# Autodesk Inventor assembly: M178-0001
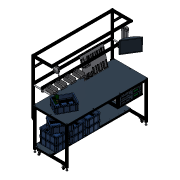
[picture p0: Inventor's stored thumbnail of the model, 180x180]
Saved by Autodesk Inventor 2018.3 (Build 223284000, 284)
## iProperties
Created: 2004-11-17
Part Number: M178-0001
Document SubType Name: Assembly
Designer: Autodesk, Inc.
Manufacturer: Standard
Standards Organization: Custom
Description: TEST STATION, STANDARD
Mass: 86518 g
Surface Area: 222281 cm^2
Volume: 49426.1 cm^3
Density: 1.75045 g/cm^3
Company: Autodesk, Inc.
Author: Autodesk, Inc.
CAGE: 1LJX3
Dept. ID: Product Design
Description #2: ---
Finish #1: ---
Finish #2: ---
Material ID: ---
Project Number: ---
## iProperties of the stored document _VirtualPart2
Created: 2006-02-28
Designer: Autodesk, Inc
Part Number: M178-S002
Description: TEST STATION SERVER SOFTWARE
Engineer: N. GINEER
Author: Autodesk, Inc
Revision Number: A
## iProperties of the stored document _VirtualPart0
Created: 2006-02-28
Part Number: E85-02674
Description: WINDOWS XP PROFESSIONAL, SP2
Designer: Autodesk, Inc
Engineer: N. GINEER
Author: Autodesk, Inc
## iProperties of the stored document _VirtualPart1
Created: 2006-02-28
Designer: Autodesk, Inc
Part Number: M178-S001
Description: TEST STATION CLIENT SOFTWARE
Engineer: N. GINEER
Author: Autodesk, Inc
Revision Number: A
## Documents named in this file (14)
- C:\AVAInvAPI\Workspace\Test Station\Test Station.iam
- C:\AVAInvAPI\Workspace\Test Station\Components\M178-1000.iam
- C:\AVAInvAPI\Workspace\Test Station\Components\M178-2000.iam
- C:\AVAInvAPI\Workspace\Test Station\Components\Standard Tote.iam
- C:\AVAInvAPI\Workspace\Test Station\Components\22-128Z2 Hardware Set.iam
- C:\AVAInvAPI\Workspace\Test Station\Components\Filled Tote 2.iam
- C:\AVAInvAPI\Workspace\Test Station\Components\22-124.ipt
- C:\AVAInvAPI\Workspace\Test Station\Components\M178-3000.iam
- C:\AVAInvAPI\Workspace\Test Station\Components\M178-4000 Phantom.iam
- C:\AVAInvAPI\Workspace\Test Station\Components\PC, RACK MOUNT, 2U.ipt
- C:\AVAInvAPI\Workspace\Test Station\Components\Monitor Phantom.iam
- C:\AVAInvAPI\Workspace\Test Station\Components\50-601.ipt
- C:\Program Files\Autodesk\Inventor 2009\Samples\Models\Assemblies\Test Station\Content\22-1x Part Bins.ipt
- C:\Program Files\Autodesk\Inventor 2009\Samples\Models\Assemblies\Test Station\Content\50-60x Zero Gravity Tool Balancer.ipt
## Components (28 placed, 14 different names)
1. M178-1000:1 [sub-assembly] — Mate:1, Flush:1, Mate:2, Mate:3, Mate:10, Flush:2, Flush:3, Mate:11
2. M178-2000:1 [sub-assembly] — Mate:1, Flush:1, Mate:2, Mate:21, Mate:22, Mate:23
3. M178-3000:1 [sub-assembly] — Mate:10, Flush:2, Flush:3, Mate:12, Mate:13, Angle:1, Mate:16, Mate:17, Angle:2, Mate:18, Mate:19, Flush:5, Mate:20, Flush:6
4. Standard Tote:14 [sub-assembly] — Mate:4
5. Filled Tote 2:1 [sub-assembly] — Mate:11
6. 50-601:1 — Mate:16, Mate:17, Angle:2
7. Monitor Phantom:1 [sub-assembly] — Mate:18, Mate:19, Flush:5
8. M178-4000 Phantom:1 [sub-assembly] — Mate:20, Flush:6
9. PC, RACK MOUNT, 2U:1 — Mate:21, Mate:22, Mate:23, Flush:7, Flush:8, Mate:24
10. PC, RACK MOUNT, 2U:2 — Flush:7, Flush:8, Mate:24
11. Windows XP Professional, SP2:1
12. Windows XP Professional, SP2:2
13. Test Station Client Software:1
14. Test Station Server Software:1
15. Standard Tote:6 [sub-assembly] — Mate:3
16. Standard Tote:7 [sub-assembly] — Mate:4
17. Standard Tote:8 [sub-assembly]
18. Standard Tote:9 [sub-assembly]
19. Standard Tote:10 [sub-assembly]
20. Standard Tote:11 [sub-assembly]
21. 22-124:1 — Mate:14, Mate:15, Flush:4
22. 22-128Z2 Hardware Set:1 [sub-assembly] — Mate:12, Mate:13, Angle:1, Mate:14, Mate:15, Flush:4
23. 22-124:2
24. 22-128Z2 Hardware Set:4 [sub-assembly]
25. 22-124:3
26. 22-128Z2 Hardware Set:5 [sub-assembly]
27. 22-124:4
28. 22-128Z2 Hardware Set:6 [sub-assembly]
## Component patterns: Totes Pattern (6 elements), (4 elements, first: 22-124:1 + 22-128Z2 Hardware Set:1)
## Relationships (29: Mate 19, Flush 8, Angle 2)
- Mate:1: M178-1000:1 ↔ M178-2000:1
- Flush:1: M178-1000:1 ↔ M178-2000:1
- Mate:2 (76.2 mm): M178-1000:1 ↔ M178-2000:1
- Mate:3: M178-1000:1 ↔ Standard Tote:6
- Mate:4: Standard Tote:14 ↔ Standard Tote:7
- Mate:10: M178-1000:1 ↔ M178-3000:1
- Flush:2: M178-1000:1 ↔ M178-3000:1
- Flush:3: M178-1000:1 ↔ M178-3000:1
- Mate:11: M178-1000:1 ↔ Filled Tote 2:1
- Mate:12: M178-3000:1 ↔ 22-128Z2 Hardware Set:1
- Mate:13 (4 mm): M178-3000:1 ↔ 22-128Z2 Hardware Set:1
- Angle:1 (0 deg): M178-3000:1 ↔ 22-128Z2 Hardware Set:1
- Mate:14: 22-124:1 ↔ 22-128Z2 Hardware Set:1
- Mate:15: 22-124:1 ↔ 22-128Z2 Hardware Set:1
- Flush:4 (-20 mm): 22-124:1 ↔ 22-128Z2 Hardware Set:1
- Angle:2 (0 deg): M178-3000:1 ↔ 50-601:1
- Mate:18: M178-3000:1 ↔ Monitor Phantom:1
- Mate:19: M178-3000:1 ↔ Monitor Phantom:1
- Flush:5 (-50.8 mm): M178-3000:1 ↔ Monitor Phantom:1
- Mate:20: M178-3000:1 ↔ M178-4000 Phantom:1
- Flush:6: M178-3000:1 ↔ M178-4000 Phantom:1
- Mate:21: M178-2000:1 ↔ PC, RACK MOUNT, 2U:1
- Mate:22: M178-2000:1 ↔ PC, RACK MOUNT, 2U:1
- Mate:23: M178-2000:1 ↔ PC, RACK MOUNT, 2U:1
- Flush:7: PC, RACK MOUNT, 2U:1 ↔ PC, RACK MOUNT, 2U:2
- Flush:8: PC, RACK MOUNT, 2U:1 ↔ PC, RACK MOUNT, 2U:2
- Mate:24: PC, RACK MOUNT, 2U:1 ↔ PC, RACK MOUNT, 2U:2
- Mate:16: M178-3000:1 ↔ 50-601:1
- Mate:17: M178-3000:1 ↔ 50-601:1
